# Autodesk Inventor assembly: mx28_withHorn
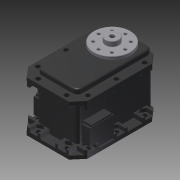
[picture p0: Inventor's stored thumbnail of the model, 180x180]
Saved by Autodesk Inventor 2016 (Build 200138000, 138)
## iProperties
Created: 2014-04-23
Part Number: mx28_withHorn
Document SubType Name: Assembly
Designer: BitBots
Mass: 44.0409 g
Surface Area: 119.943 cm^2
Volume: 44.0409 cm^3
Density: 1 g/cm^3
Author: BitBots
## Documents named in this file (3)
- Z:\nimbro_cad\NICU_Assembly_CAD\arms_new\motors\Mx28\mx28_with_horn.iam
- Z:\nimbro_cad\NICU_Assembly_CAD\motors_new\Mx28\Imported Components\RX-28\RX-28.ipt
- Z:\nimbro_cad\NICU_Assembly_CAD\arms_new\Imported Components\HN07-N101\HN07-N101.ipt
## Components (2 placed, 2 different names)
1. RX-28:1 — Rotational:2
2. HN07-N101:1 — Rotational:2
## Relationships (1: RevoluteJoint 1)
- Rotational:2 [RevoluteJoint]: RX-28:1 ↔ HN07-N101:1
